# Autodesk Inventor assembly: feb 22 assemblying
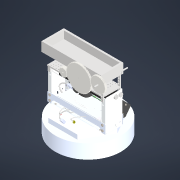
[picture p0: Inventor's stored thumbnail of the model, 180x180]
Saved by Autodesk Inventor 2021 (Build 250183000, 183)
## iProperties
Created: 2021-01-23
Part Number: feb 22 assemblying
Document SubType Name: Assembly
Designer: benji
Author: benji
## Documents named in this file (11)
- C:\Users\benji\OneDrive\Neil Lauren Benji Emma shared\Benji McMaster\2021 Winter Term\Engineering 1P13B\project 3 cad files\P3 early playing around\feb 22 assemblying.iam
- C:\Users\benji\OneDrive\Neil Lauren Benji Emma shared\Benji McMaster\2021 Winter Term\Engineering 1P13B\project 3 cad files\Rotary Actuator\Stepper Motor.iam
- C:\Users\benji\OneDrive\Neil Lauren Benji Emma shared\Benji McMaster\2021 Winter Term\Engineering 1P13B\project 3 cad files\Q-Bot baseplate\Mounting Platform.iam
- C:\Users\benji\OneDrive\Neil Lauren Benji Emma shared\Benji McMaster\2021 Winter Term\Engineering 1P13B\project 3 cad files\Q-Bot Assembly\QBot.iam
- C:\Users\benji\OneDrive\Neil Lauren Benji Emma shared\Benji McMaster\2021 Winter Term\Engineering 1P13B\project 3 cad files\GivenHopper (to be modified by your team).ipt
- C:\Users\benji\OneDrive\Neil Lauren Benji Emma shared\Benji McMaster\2021 Winter Term\Engineering 1P13B\project 3 cad files\P3 early playing around\hopper hole rod.ipt
- C:\Users\benji\OneDrive\Neil Lauren Benji Emma shared\Benji McMaster\2021 Winter Term\Engineering 1P13B\project 3 cad files\P3 early playing around\gudGearsAttempt1\Design Accelerator\Spur Gear11.ipt
- C:\Users\benji\OneDrive\Neil Lauren Benji Emma shared\Benji McMaster\2021 Winter Term\Engineering 1P13B\project 3 cad files\P3 early playing around\gudGearsAttempt1.5\Design Accelerator\Spur Gear11.ipt
- C:\Users\benji\OneDrive\Neil Lauren Benji Emma shared\Benji McMaster\2021 Winter Term\Engineering 1P13B\project 3 cad files\P3 early playing around\gudGearsAttempt1\Design Accelerator\Spur Gear21.ipt
- C:\Users\benji\OneDrive\Neil Lauren Benji Emma shared\Benji McMaster\2021 Winter Term\Engineering 1P13B\project 3 cad files\P3 early playing around\gud gear stand proto 1 2.ipt
- C:\Users\benji\OneDrive\Neil Lauren Benji Emma shared\Benji McMaster\2021 Winter Term\Engineering 1P13B\project 3 cad files\P3 early playing around\linkage connector proto 1.ipt
## Components (12 placed, 9 different names)
1. Mounting Platform:1 [sub-assembly] — Mate:31, Mate:32, Angle:1, Mate:35, Mate:36, Mate:47, Mate:52, Mate:53, Flush:8, Mate:74, Mate:75, Mate:80
2. QBot:1 [sub-assembly] — Mate:31, Mate:32, Angle:1
3. GivenHopper (to be modified by your team):1 — Mate:35, Mate:36, Angle:4, Mate:68, Rotation:15, Mate:72, Mate:78
4. Stepper Motor:5 [sub-assembly] — Mate:47, Mate:52, Mate:53, Angle:4, Mate:69, Mate:73, Rotation:21
5. hopper hole rod:1 — Mate:68, Flush:8, Rotation:15, Mate:71, Rotation:16, Mate:79
6. Spur Gear1:1 — Mate:69, Mate:73, Flush:9, Rotation:19, Rotation:21
7. Spur Gear1:2 — Mate:71, Mate:72, Rotation:16, Rotation:20
8. Spur Gear2:1 — Flush:9, Mate:76, Rotation:19, Rotation:20
9. gud gear stand proto 1 2:1 — Mate:74, Mate:75, Mate:76, Mate:77
10. Spur Gear2:2 — Mate:77, Mate:78, Flush:10
11. Spur Gear1:3 — Mate:79, Flush:10
12. linkage connector proto 1:1 — Mate:80
## Relationships (29: Mate 19, RelateRotation 5, Flush 3, Angle 2)
- Mate:31: Mounting Platform:1 ↔ QBot:1
- Mate:32: Mounting Platform:1 ↔ QBot:1
- Angle:1 (0 deg): Mounting Platform:1 ↔ QBot:1
- Mate:35: Mounting Platform:1 ↔ GivenHopper (to be modified by your team):1
- Mate:36 (0.224 mm): Mounting Platform:1 ↔ GivenHopper (to be modified by your team):1
- Mate:47: Mounting Platform:1 ↔ Stepper Motor:5
- Mate:52: Mounting Platform:1 ↔ Stepper Motor:5
- Mate:53: Mounting Platform:1 ↔ Stepper Motor:5
- Angle:4 (120 deg): GivenHopper (to be modified by your team):1 ↔ Stepper Motor:5
- Mate:68: GivenHopper (to be modified by your team):1 ↔ hopper hole rod:1
- Flush:8 (-41.189 mm): Mounting Platform:1 ↔ hopper hole rod:1
- Rotation:15 [RelateRotation] (1 ul): GivenHopper (to be modified by your team):1 ↔ hopper hole rod:1
- Mate:69: Stepper Motor:5 ↔ Spur Gear1:1
- Mate:71: hopper hole rod:1 ↔ Spur Gear1:2
- Mate:72: GivenHopper (to be modified by your team):1 ↔ Spur Gear1:2
- Rotation:16 [RelateRotation] (1 ul): hopper hole rod:1 ↔ Spur Gear1:2
- Mate:73 (1.1 mm): Stepper Motor:5 ↔ Spur Gear1:1
- Flush:9 (-0.5 mm): Spur Gear1:1 ↔ Spur Gear2:1
- Mate:74: Mounting Platform:1 ↔ gud gear stand proto 1 2:1
- Mate:75: Mounting Platform:1 ↔ gud gear stand proto 1 2:1
- Mate:76: Spur Gear2:1 ↔ gud gear stand proto 1 2:1
- Rotation:19 [RelateRotation] (0.3077 ul): Spur Gear1:1 ↔ Spur Gear2:1
- Rotation:20 [RelateRotation] (1.6774 ul): Spur Gear1:2 ↔ Spur Gear2:1
- Rotation:21 [RelateRotation] (1 ul): Stepper Motor:5 ↔ Spur Gear1:1
- Mate:77: gud gear stand proto 1 2:1 ↔ Spur Gear2:2
- Mate:78: GivenHopper (to be modified by your team):1 ↔ Spur Gear2:2
- Mate:79: hopper hole rod:1 ↔ Spur Gear1:3
- Flush:10: Spur Gear2:2 ↔ Spur Gear1:3
- Mate:80: Mounting Platform:1 ↔ linkage connector proto 1:1
